# Autodesk Inventor assembly: WS2017_M3508_______ASM
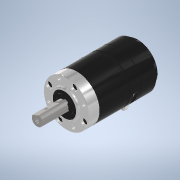
[picture p0: Inventor's stored thumbnail of the model, 180x180]
Saved by Autodesk Inventor 2020.2 (Build 242310000, 310)
## iProperties
Created: 2019-05-05
Part Number: WS2017_M3508_______ASM
Document SubType Name: Assembly
Designer: boxi
Author: boxi
Revision Number: 2LAST_VERSION
## Documents named in this file (7)
- C:\Users\boxi\Documents\flexipod_hardware\mechanical_model\motor_DJI_M3508\motor_DJI_M3508.iam
- C:\Users\boxi\Documents\flexipod_hardware\mechanical_model\motor_DJI_M3508\4_ASM.iam
- C:\Users\boxi\Documents\flexipod_hardware\mechanical_model\motor_DJI_M3508\5_ASM.iam
- C:\Users\boxi\Documents\flexipod_hardware\mechanical_model\motor_DJI_M3508\1_1.ipt
- C:\Users\boxi\Documents\flexipod_hardware\mechanical_model\motor_DJI_M3508\3.ipt
- C:\Users\boxi\Documents\flexipod_hardware\mechanical_model\motor_DJI_M3508\2_ASM.iam
- C:\Users\boxi\Documents\flexipod_hardware\mechanical_model\motor_DJI_M3508\17.ipt
## Components (6 placed, 6 different names)
1. 4 [sub-assembly]
2. 10 [sub-assembly]
3. 11
4. 12
5. 27 [sub-assembly] — Mate:1, Mate:2
6. 15 — Mate:1, Mate:2
## Relationships (2: Mate 2)
- Mate:1: 27 ↔ 15
- Mate:2: 27 ↔ 15
